# Autodesk Inventor assembly: Proper
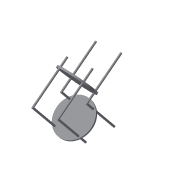
[picture p0: Inventor's stored thumbnail of the model, 180x180]
Saved by Autodesk Inventor 2017 (Build 210142000, 142)
## iProperties
Created: 2019-06-26
Part Number: Proper
Document SubType Name: Assembly
Designer: Admin
Author: Admin
## Documents named in this file (5)
- E:\8 mechanism\1\Right angle\Proper.iam
- E:\8 mechanism\1\Right angle\Part1.ipt
- E:\8 mechanism\1\Right angle\Part3.ipt
- E:\8 mechanism\1\Right angle\Part4.ipt
- E:\8 mechanism\1\Right angle\Part5.ipt
## Components (9 placed, 4 different names)
1. Part1:1 — Angle:1, Tangent:2, Mate:8, Mate:10, Mate:11, Mate:14, Rotational:1
2. Part3:1 — Rotational:1
3. Part3:2 — Mate:2, Mate:4
4. Part4:1 — Mate:13, Mate:14
5. Part1:2 — Mate:2, Mate:4, Angle:1, Tangent:1, Mate:7, Mate:9, Mate:12, Mate:13
6. Part5:1 — Tangent:1, Tangent:2
7. Part4:2 — Mate:7, Mate:8
8. Part4:3 — Mate:9, Mate:10
9. Part4:4 — Mate:11, Mate:12
## Relationships (14: Mate 10, Tangent 2, Angle 1, RevoluteJoint 1)
- Mate:2: Part3:2 ↔ Part1:2
- Mate:4: Part3:2 ↔ Part1:2
- Angle:1 (90 deg): Part1:1 ↔ Part1:2
- Tangent:1: Part1:2 ↔ Part5:1
- Tangent:2: Part1:1 ↔ Part5:1
- Mate:7: Part1:2 ↔ Part4:2
- Mate:8: Part1:1 ↔ Part4:2
- Mate:9: Part1:2 ↔ Part4:3
- Mate:10: Part1:1 ↔ Part4:3
- Mate:11: Part1:1 ↔ Part4:4
- Mate:12: Part1:2 ↔ Part4:4
- Mate:13: Part4:1 ↔ Part1:2
- Mate:14: Part1:1 ↔ Part4:1
- Rotational:1 [RevoluteJoint]: Part1:1 ↔ Part3:1
